# Autodesk Inventor assembly: wheel1
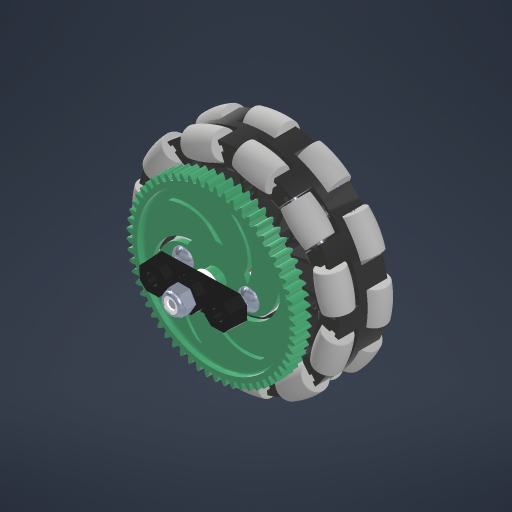
[picture p0: Inventor's stored thumbnail of the model, 512x512]
Saved by Autodesk Inventor 2024 (Build 280153000, 153)
## iProperties
Created: 2023-08-09
Part Number: wheel1
Document SubType Name: Assembly
Designer: macbook
Author: macbook
## Documents named in this file (13)
- \\Mac\Home\Desktop\code\1599V-VRC\Cad\Assembly\v3\omniwheel.iam
- \\Mac\Home\Desktop\code\1599V-VRC\Cad\Motion\Shaft LS\Bearing Flat.ipt
- \\Mac\Home\Desktop\code\1599V-VRC\Cad\Structure\Hardware\Nut Nylock.ipt
- \\Mac\Home\Desktop\code\1599V-VRC\Cad\Structure\Hardware\Screw Steel - Star\SScrew Star Smooth 2.500.ipt
- \\Mac\Home\Desktop\code\1599V-VRC\Cad\Motion\Gears\LS 60T Gear.ipt
- \\Mac\Home\Desktop\code\1599V-VRC\Cad\Structure\Hardware\Screw Steel - Star\SScrew Star Threaded 1.250.ipt
- \\Mac\Home\Desktop\code\1599V-VRC\Cad\Motion\Spacers\Spacer Nylon .500 OD\NSpacer White .500 OD x .375.ipt
- \\Mac\Home\Desktop\code\1599V-VRC\Cad\Motion\Spacers\Spacer Nylon .500 OD\NSpacer White .500 OD x .500.ipt
- \\Mac\Home\Desktop\code\1599V-VRC\Cad\Motion\Wheels\Omni Wheel\3.25 Omni AS, cir.iam
- \\Mac\Home\Desktop\code\1599V-VRC\Cad\Structure\Hardware\Screw Steel - Star.ipt
- \\Mac\Home\Desktop\code\1599V-VRC\Cad\Motion\Spacers\Spacer Nylon .500 OD.ipt
- \\Mac\Home\Desktop\code\1599V-VRC\Cad\Motion\Spacers\Washer Teflon.ipt
- \\Mac\Home\Desktop\code\1599V-VRC\Cad\Motion\Spacers\Washer Teflon\TWasher .375 OD x .06250.ipt
## Components (15 placed, 9 different names)
1. 3.25 Omni AS, cir:3 [sub-assembly] — Insert:117, Insert:118, Insert:130, Insert:131, Insert:132
2. Nut Nylock:10 — Insert:117
3. Nut Nylock:11 — Insert:118
4. Bearing Flat:6
5. Bearing Flat:7 — Insert:134
6. SScrew Star Smooth 2.500:18
7. Nut Nylock:12
8. NSpacer White .500 OD x .500:11 — Insert:132, Insert:133
9. LS 60T Gear:2 — Insert:127, Insert:128, Insert:129, Insert:135
10. NSpacer White .500 OD x .375:12 — Insert:129, Insert:130
11. NSpacer White .500 OD x .375:13 — Insert:131
12. SScrew Star Threaded 1.250:19 — Insert:127
13. SScrew Star Threaded 1.250:20 — Insert:128
14. TWasher .375 OD x .06250:1 — Insert:133, Insert:134
15. TWasher .375 OD x .06250:2 — Insert:135
## Relationships (16: Insert 16)
- Insert:117: 3.25 Omni AS, cir:3 ↔ Nut Nylock:10
- Insert:118: 3.25 Omni AS, cir:3 ↔ Nut Nylock:11
- [Insert] (44.45 mm): Bearing Flat:6 ↔ Bearing Flat:7
- [Insert] (44.45 mm): Bearing Flat:6 ↔ Bearing Flat:7
- [Insert] (1.5875 mm): Bearing Flat:7 ↔ SScrew Star Smooth 2.500:18
- [Insert]: Bearing Flat:6 ↔ Nut Nylock:12
- [Insert]: LS 60T Gear:2 ↔ NSpacer White .500 OD x .375:13
- Insert:127: LS 60T Gear:2 ↔ SScrew Star Threaded 1.250:19
- Insert:128: LS 60T Gear:2 ↔ SScrew Star Threaded 1.250:20
- Insert:129: LS 60T Gear:2 ↔ NSpacer White .500 OD x .375:12
- Insert:130: 3.25 Omni AS, cir:3 ↔ NSpacer White .500 OD x .375:12
- Insert:131: 3.25 Omni AS, cir:3 ↔ NSpacer White .500 OD x .375:13
- Insert:132: 3.25 Omni AS, cir:3 ↔ NSpacer White .500 OD x .500:11
- Insert:133: NSpacer White .500 OD x .500:11 ↔ TWasher .375 OD x .06250:1
- Insert:134: Bearing Flat:7 ↔ TWasher .375 OD x .06250:1
- Insert:135: LS 60T Gear:2 ↔ TWasher .375 OD x .06250:2
## Named parameters: d125_d111_d47 = 44.45 mm, d126_d112_d48 = 44.45 mm, d127_d113_d71 = 1.5875 mm, d128_d114_d72 = 0 mm, d132_d92 = 0 mm
